# Autodesk Inventor assembly: Frame
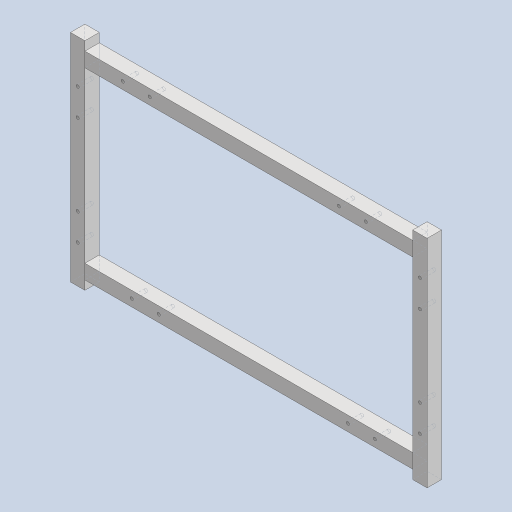
[picture p0: Inventor's stored thumbnail of the model, 512x512]
Saved by Autodesk Inventor 2023.4 (Build 274418000, 418)
## iProperties
Created: 2024-02-16
Part Number: Frame
Document SubType Name: Assembly
Designer: PalumaCMM
Author: PalumaCMM
## Documents named in this file (3)
- C:\Users\PalumaCMM\Documents\Inventor\Sucharitha\Frame\Frame.iam
- C:\Users\PalumaCMM\Documents\Inventor\Sucharitha\Frame\Long side frame.ipt
- C:\Users\PalumaCMM\Documents\Inventor\Sucharitha\Frame\Shorter side frame.ipt
## Components (4 placed, 2 different names)
1. Long side frame:1 — Flush:2, Flush:7, Flush:8, Mate:1
2. Shorter side frame:1 — Flush:1, Flush:2, Flush:6, Flush:8, Mate:1, Mate:3
3. Long side frame:2 — Flush:1, Flush:3, Flush:6, Mate:2, Mate:3
4. Shorter side frame:2 — Flush:3, Flush:7, Mate:2
## Relationships (9: Flush 6, Mate 3)
- Flush:1: Shorter side frame:1 ↔ Long side frame:2
- Flush:2: Long side frame:1 ↔ Shorter side frame:1
- Flush:3: Long side frame:2 ↔ Shorter side frame:2
- Flush:6 (25 mm): Shorter side frame:1 ↔ Long side frame:2
- Flush:7 (-25 mm): Long side frame:1 ↔ Shorter side frame:2
- Flush:8 (-25 mm): Long side frame:1 ↔ Shorter side frame:1
- Mate:1: Long side frame:1 ↔ Shorter side frame:1
- Mate:2: Long side frame:2 ↔ Shorter side frame:2
- Mate:3: Shorter side frame:1 ↔ Long side frame:2
